# Autodesk Inventor assembly: Actuador sin carro
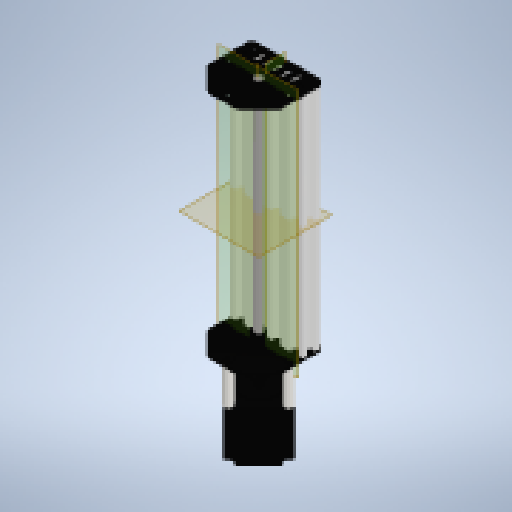
[picture p0: Inventor's stored thumbnail of the model, 512x512]
Saved by Autodesk Inventor 2024.2 (Build 282272000, 272)
## iProperties
Created: 2023-12-09
Part Number: Actuador sin carro
Document SubType Name: Assembly
Designer: juanp
Author: juanp
## Documents named in this file (26)
- C:\Users\jp.reyesf\OneDrive - Universidad de los andes\Uniandes\GPR Portable\Actuador\Actuador Lineal NEMA23\Actuador sin carro.iam
- C:\Users\jp.reyesf\OneDrive - Universidad de los andes\Uniandes\GPR Portable\Actuador\Actuador Lineal NEMA23\Solid1.ipt
- C:\Users\jp.reyesf\OneDrive - Universidad de los andes\Uniandes\GPR Portable\Actuador\Actuador Lineal NEMA23\Solid2.ipt
- C:\Users\jp.reyesf\OneDrive - Universidad de los andes\Uniandes\GPR Portable\Actuador\Actuador Lineal NEMA23\Solid35.ipt
- C:\Users\jp.reyesf\OneDrive - Universidad de los andes\Uniandes\GPR Portable\Actuador\Actuador Lineal NEMA23\Solid36.ipt
- C:\Users\jp.reyesf\OneDrive - Universidad de los andes\Uniandes\GPR Portable\Actuador\Actuador Lineal NEMA23\Solid37.ipt
- C:\Users\jp.reyesf\OneDrive - Universidad de los andes\Uniandes\GPR Portable\Actuador\Actuador Lineal NEMA23\Solid38.ipt
- C:\Users\jp.reyesf\OneDrive - Universidad de los andes\Uniandes\GPR Portable\Actuador\Actuador Lineal NEMA23\Solid39.ipt
- C:\Users\jp.reyesf\OneDrive - Universidad de los andes\Uniandes\GPR Portable\Actuador\Actuador Lineal NEMA23\Solid40.ipt
- C:\Users\jp.reyesf\OneDrive - Universidad de los andes\Uniandes\GPR Portable\Actuador\Actuador Lineal NEMA23\Solid41.ipt
- C:\Users\jp.reyesf\OneDrive - Universidad de los andes\Uniandes\GPR Portable\Actuador\Actuador Lineal NEMA23\Solid42.ipt
- C:\Users\jp.reyesf\OneDrive - Universidad de los andes\Uniandes\GPR Portable\Actuador\Actuador Lineal NEMA23\Solid43.ipt
- C:\Users\jp.reyesf\OneDrive - Universidad de los andes\Uniandes\GPR Portable\Actuador\Actuador Lineal NEMA23\Solid44.ipt
- C:\Users\jp.reyesf\OneDrive - Universidad de los andes\Uniandes\GPR Portable\Actuador\Actuador Lineal NEMA23\Solid45.ipt
- C:\Users\jp.reyesf\OneDrive - Universidad de los andes\Uniandes\GPR Portable\Actuador\Actuador Lineal NEMA23\Solid46.ipt
- C:\Users\jp.reyesf\OneDrive - Universidad de los andes\Uniandes\GPR Portable\Actuador\Actuador Lineal NEMA23\Solid47.ipt
- C:\Users\jp.reyesf\OneDrive - Universidad de los andes\Uniandes\GPR Portable\Actuador\Actuador Lineal NEMA23\Solid48.ipt
- C:\Users\jp.reyesf\OneDrive - Universidad de los andes\Uniandes\GPR Portable\Actuador\Actuador Lineal NEMA23\Solid49.ipt
- C:\Users\jp.reyesf\OneDrive - Universidad de los andes\Uniandes\GPR Portable\Actuador\Actuador Lineal NEMA23\Solid50.ipt
- C:\Users\jp.reyesf\OneDrive - Universidad de los andes\Uniandes\GPR Portable\Actuador\Actuador Lineal NEMA23\Solid51.ipt
- C:\Users\jp.reyesf\OneDrive - Universidad de los andes\Uniandes\GPR Portable\Actuador\Actuador Lineal NEMA23\Solid52.ipt
- C:\Users\jp.reyesf\OneDrive - Universidad de los andes\Uniandes\GPR Portable\Actuador\Actuador Lineal NEMA23\Solid53.ipt
- C:\Users\jp.reyesf\OneDrive - Universidad de los andes\Uniandes\GPR Portable\Actuador\Actuador Lineal NEMA23\Solid66.ipt
- C:\Users\jp.reyesf\OneDrive - Universidad de los andes\Uniandes\GPR Portable\Actuador\Actuador Lineal NEMA23\Solid67.ipt
- C:\Users\jp.reyesf\OneDrive - Universidad de los andes\Uniandes\GPR Portable\Actuador\Actuador Lineal NEMA23\Solid68.ipt
- C:\Users\jp.reyesf\OneDrive - Universidad de los andes\Uniandes\GPR Portable\Actuador\Actuador Lineal NEMA23\Solid69.ipt
## Components (25 placed, 25 different names)
1. Solid1:1
2. Solid2:1
3. Solid35:1 — Mate:1
4. Solid36:1
5. Solid37:1
6. Solid38:1
7. Solid39:1
8. Solid40:1
9. Solid41:1
10. Solid42:1
11. Solid43:1
12. Solid44:1
13. Solid45:1 — Symmetry:1
14. Solid46:1 — Symmetry:1
15. Solid47:1 — Angle:1, Angle:2
16. Solid48:1
17. Solid49:1
18. Solid50:1
19. Solid51:1
20. Solid52:1
21. Solid53:1
22. Solid66:1
23. Solid67:1
24. Solid68:1
25. Solid69:1
## Relationships (6: Mate 3, Angle 2, Symmetry 1)
- Symmetry:1: Solid45:1 ↔ Solid46:1
- Mate:1: Solid35:1
- Mate:2
- Angle:1 (90 deg): Solid47:1
- Mate:3
- Angle:2 (0 deg): Solid47:1
